# Autodesk Inventor assembly: C-SHA30
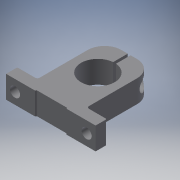
[picture p0: Inventor's stored thumbnail of the model, 180x180]
Saved by Autodesk Inventor 2019 (Build 230136000, 136)
## iProperties
Category: PARTsolutions
Company: MISUMI
Created: 2022-11-16
Part Number: C-SHA30
Catalog Web Link: www.cadenas.de
Description: C-SHA-Economy Shaft Supports - T-Shaped/Slit
Vendor: MISUMI
Document SubType Name: Assembly
Designer: psAdmin
Manufacturer: MISUMI
Mass: 49.6366 g
Surface Area: 148.895 cm^2
Volume: 49.6366 cm^3
Density: 1 g/cm^3
Title: C-SHA30
Author: Cadenas PARTsolutions
Comments: Economy Shaft Supports - T-Shaped/Slit
PSOL_IDENT_0: {$CADENAS_DATA/23d-libs/misumi/metric/02_shaft_supports/c_sha_asmtab.prj},167 {VTYP=3D},{STYP=ASSTAB
PSOL_IDENT_1: },{NB=C-SHA30},{LINA=C-SHA30},{NN=C-SHA},{DATE=04.10.2022 06:54:20},{GEOMDATE=23.04.2021 02:50:35},{
PSOL_IDENT_2: VERSION=},{LINEID=60},{WBVAR=},{WBNUMERIC=}  {NB=C-SHA30},{LINA=C-SHA30},{KT=DUMMY},{PN=C-SHA30},{TY
PSOL_IDENT_3: PE=C-SHA},{D=30},{H=42},{H1=70},{T=20},{L1=64},{DD=9.0},{E=21.0},{S=10},{R=15},{L=80},{B=28},{W=44},
PSOL_IDENT_4: {M=M6},{R2=2},{W2=2.5},{M3D=6},{M3D2=13.5},{M3D3=11},{M3D4=6.4},{LB=20},{PPATH=c_sha/c_sha_asmtpl.pr
PSOL_IDENT_5: j}
NB: C-SHA30
NN: C-SHA
NT: Economy Shaft Supports - T-Shaped/Slit
NBSYN: $PN.
LINA: C-SHA30
CATALOG: Misumi
PN: C-SHA30
D: 30
H: 42
H1: 70
T: 20
L1: 64
DD: 9
E: 21
S: 10
R: 15
L: 80
B: 28
W: 44
M: M6
SUPPLIER: MISUMI
ARTICLENO: C-SHA30
BOMINFO: C-SHA30
CREATOR: CADENAS GmbH
## Documents named in this file (3)
- e:\temp\worker_COMMON_2\temp\tmp_720_120_UZ9P2\format_0\C-SHA30.iam
- e:\temp\worker_COMMON_2\temp\tmp_720_120_UZ9P2\format_0\C-SHA30_b.ipt
- e:\temp\worker_COMMON_2\temp\tmp_720_120_UZ9P2\format_0\BOLT6-20.ipt
## Components (2 placed, 2 different names)
1. C-SHA30_b:1 — to_bolt_XY@1 <-> to_cp_XY@2, to_bolt_Z@1 <-> to_cp_Z@2, to_bolt_YZ@1 <-> to_cp_YZ@2
2. BOLT6-20:1 — to_bolt_XY@1 <-> to_cp_XY@2, to_bolt_Z@1 <-> to_cp_Z@2, to_bolt_YZ@1 <-> to_cp_YZ@2
## Relationships (3: Mate 2, Angle 1)
- to_bolt_XY@1 <-> to_cp_XY@2 [Mate]: C-SHA30_b:1 ↔ BOLT6-20:1
- to_bolt_Z@1 <-> to_cp_Z@2 [Mate]: C-SHA30_b:1 ↔ BOLT6-20:1
- to_bolt_YZ@1 <-> to_cp_YZ@2 [Angle] (0 deg): C-SHA30_b:1 ↔ BOLT6-20:1
